# Autodesk Inventor assembly: Laser
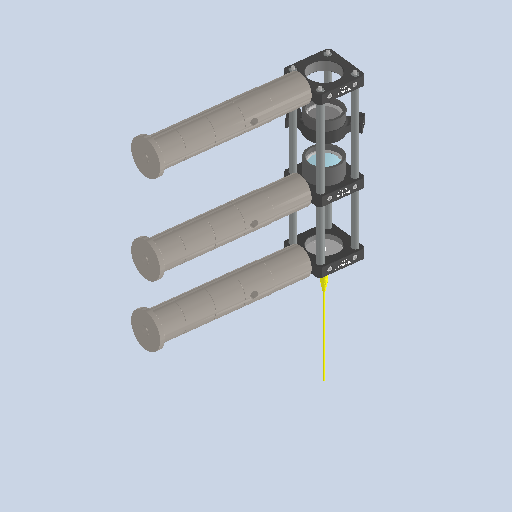
[picture p0: Inventor's stored thumbnail of the model, 512x512]
Saved by Autodesk Inventor 2026.1 (Build 301233000, 233)
## iProperties
Created: 2025-05-29
Part Number: Laser
Document SubType Name: Assembly
Designer: Julian
Author: Julian
## Documents named in this file (9)
- C:\Users\user\Desktop\setup_inventor_2025\anregung\Laser.iam
- C:\Users\user\Desktop\setup_inventor_2025\anregung\CP33_M_no tings.ipt
- C:\Users\user\Desktop\setup_inventor_2025\anregung\AC254-060-A-ML-Step.ipt
- C:\Users\user\Desktop\setup_inventor_2025\anregung\SM1FCA-Step.ipt
- C:\Users\user\Desktop\setup_inventor_2025\anregung\P1-S405Y-FC-1-Step.ipt
- C:\Users\user\Desktop\setup_inventor_2025\anregung\Newport-M-PS-4.ipt
- C:\Users\user\Desktop\setup_inventor_2025\anregung\ER6-Step.ipt
- C:\Users\user\Desktop\setup_inventor_2025\anregung\NE10A-A-Step.ipt
- C:\Users\user\Desktop\setup_inventor_2025\anregung\DCP1.ipt
## Components (15 placed, 8 different names)
1. CP33_M_no tings:1 — Passend:8, Passend:9, Passend:14, Passend:17, Passend:18, Passend:21, Fluchtend:2, Fluchtend:3, Fluchtend:4, Fluchtend:5
2. CP33_M_no tings:2 — Passend:1, Passend:2, Passend:7, Passend:11, Passend:13, Passend:15, Passend:20, Passend:23, Passend:29
3. CP33_M_no tings:3 — Passend:3, Fluchtend:1, Passend:6, Passend:10, Passend:12, Passend:16, Passend:19, Passend:22, Fluchtend:6, Fluchtend:7, Fluchtend:8, Fluchtend:9
4. AC254-060-A-ML-Step:1 — Passend:1, Passend:2, Passend:24
5. SM1FCA-Step:1 — Passend:3, Fluchtend:1, Passend:4, Passend:5, Passend:24
6. P1-S405Y-FC-1-Step:1 — Passend:4, Passend:5
7. Newport-M-PS-4:1 — Passend:7, Passend:11
8. Newport-M-PS-4:2 — Passend:6, Passend:10
9. Newport-M-PS-4:3 — Passend:8, Passend:9
10. ER6-Step:1 — Passend:21, Passend:22, Passend:23, Fluchtend:2, Fluchtend:7
11. ER6-Step:2 — Passend:18, Passend:19, Passend:20, Fluchtend:4, Fluchtend:6, Passend:27
12. ER6-Step:3 — Passend:12, Passend:13, Passend:14, Fluchtend:5, Fluchtend:8
13. ER6-Step:4 — Passend:15, Passend:16, Passend:17, Fluchtend:3, Fluchtend:9, Passend:28
14. NE10A-A-Step:1 — Passend:25, Passend:26
15. DCP1:1 — Passend:25, Passend:26, Passend:27, Passend:28, Passend:29
## Relationships (38: Mate 29, Flush 9)
- Passend:1 [Mate]: CP33_M_no tings:2 ↔ AC254-060-A-ML-Step:1
- Passend:2 [Mate]: CP33_M_no tings:2 ↔ AC254-060-A-ML-Step:1
- Passend:3 [Mate]: CP33_M_no tings:3 ↔ SM1FCA-Step:1
- Fluchtend:1 [Flush] (-2 mm): CP33_M_no tings:3 ↔ SM1FCA-Step:1
- Passend:4 [Mate]: SM1FCA-Step:1 ↔ P1-S405Y-FC-1-Step:1
- Passend:5 [Mate] (6 mm): SM1FCA-Step:1 ↔ P1-S405Y-FC-1-Step:1
- Passend:6 [Mate]: CP33_M_no tings:3 ↔ Newport-M-PS-4:2
- Passend:7 [Mate]: CP33_M_no tings:2 ↔ Newport-M-PS-4:1
- Passend:8 [Mate]: CP33_M_no tings:1 ↔ Newport-M-PS-4:3
- Passend:9 [Mate]: CP33_M_no tings:1 ↔ Newport-M-PS-4:3
- Passend:10 [Mate]: CP33_M_no tings:3 ↔ Newport-M-PS-4:2
- Passend:11 [Mate]: CP33_M_no tings:2 ↔ Newport-M-PS-4:1
- Passend:12 [Mate]: CP33_M_no tings:3 ↔ ER6-Step:3
- Passend:13 [Mate]: CP33_M_no tings:2 ↔ ER6-Step:3
- Passend:14 [Mate]: CP33_M_no tings:1 ↔ ER6-Step:3
- Passend:15 [Mate]: CP33_M_no tings:2 ↔ ER6-Step:4
- Passend:16 [Mate]: CP33_M_no tings:3 ↔ ER6-Step:4
- Passend:17 [Mate]: CP33_M_no tings:1 ↔ ER6-Step:4
- Passend:18 [Mate]: CP33_M_no tings:1 ↔ ER6-Step:2
- Passend:19 [Mate]: CP33_M_no tings:3 ↔ ER6-Step:2
- Passend:20 [Mate]: CP33_M_no tings:2 ↔ ER6-Step:2
- Passend:21 [Mate]: CP33_M_no tings:1 ↔ ER6-Step:1
- Passend:22 [Mate]: CP33_M_no tings:3 ↔ ER6-Step:1
- Passend:23 [Mate]: CP33_M_no tings:2 ↔ ER6-Step:1
- Fluchtend:2 [Flush]: CP33_M_no tings:1 ↔ ER6-Step:1
- Fluchtend:3 [Flush]: CP33_M_no tings:1 ↔ ER6-Step:4
- Fluchtend:4 [Flush]: CP33_M_no tings:1 ↔ ER6-Step:2
- Fluchtend:5 [Flush]: CP33_M_no tings:1 ↔ ER6-Step:3
- Fluchtend:6 [Flush]: CP33_M_no tings:3 ↔ ER6-Step:2
- Fluchtend:7 [Flush]: CP33_M_no tings:3 ↔ ER6-Step:1
- Fluchtend:8 [Flush]: CP33_M_no tings:3 ↔ ER6-Step:3
- Fluchtend:9 [Flush]: CP33_M_no tings:3 ↔ ER6-Step:4
- Passend:24 [Mate] (60 mm): AC254-060-A-ML-Step:1 ↔ SM1FCA-Step:1
- Passend:25 [Mate]: NE10A-A-Step:1 ↔ DCP1:1
- Passend:26 [Mate]: NE10A-A-Step:1 ↔ DCP1:1
- Passend:27 [Mate]: ER6-Step:2 ↔ DCP1:1
- Passend:28 [Mate] (0.4 mm): ER6-Step:4 ↔ DCP1:1
- Passend:29 [Mate] (35 mm): CP33_M_no tings:2 ↔ DCP1:1
